# Autodesk Inventor assembly: H3-MOD-OCT2017
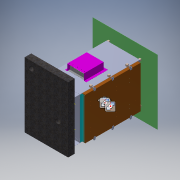
[picture p0: Inventor's stored thumbnail of the model, 180x180]
Saved by Autodesk Inventor 2017 (Build 210142000, 142)
## iProperties
Created: 2017-10-03
Part Number: H3-MOD-OCT2017
Document SubType Name: Assembly
Designer: Kathryn Rosie
Author: Kathryn Rosie
## Documents named in this file (4)
- C:\Users\Kathryn Rosie\Google Drive\HERA\hera-cad\Node\20171003\Enclosure\H3-MOD-OCT2017.iam
- C:\Users\Kathryn Rosie\Google Drive\HERA\hera-cad\Node\plinth.ipt
- C:\Users\Kathryn Rosie\Google Drive\HERA\hera-cad\Node\20171003\Enclosure\EnclosureAssy.iam
- C:\Users\Kathryn Rosie\Google Drive\HERA\hera-cad\Node\rackAssembly.iam
## Components (3 placed, 3 different names)
1. plinth:1 — Mate:1, Mate:2, Mate:3, Mate:4
2. EnclosureAssy:1 [sub-assembly] — Mate:1, Mate:2, Mate:3, Mate:4, Mate:5, Angle:1, Mate:6, Mate:7
3. rackAssembly:1 [sub-assembly] — Mate:5, Angle:1, Mate:6, Mate:7
## Relationships (8: Mate 7, Angle 1)
- Mate:1 (-80 mm): plinth:1 ↔ EnclosureAssy:1
- Mate:2 (-80 mm): plinth:1 ↔ EnclosureAssy:1
- Mate:3 (-100 mm): plinth:1 ↔ EnclosureAssy:1
- Mate:4: plinth:1 ↔ EnclosureAssy:1
- Mate:5: EnclosureAssy:1 ↔ rackAssembly:1
- Angle:1 (0 deg): EnclosureAssy:1 ↔ rackAssembly:1
- Mate:6 (150 mm): EnclosureAssy:1 ↔ rackAssembly:1
- Mate:7: EnclosureAssy:1 ↔ rackAssembly:1
